# Autodesk Inventor assembly: ForeArm
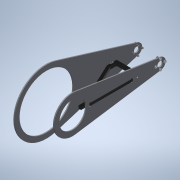
[picture p0: Inventor's stored thumbnail of the model, 180x180]
Saved by Autodesk Inventor 2020.4 (Build 244396000, 396)
## iProperties
Created: 2016-05-04
Part Number: ForeArm
Document SubType Name: Assembly
Designer: hiroaki
Mass: 49.3377 g
Surface Area: 202.128 cm^2
Volume: 30.5225 cm^3
Density: 1.61644 g/cm^3
Author: hiroaki
## Documents named in this file (5)
- C:\Users\Masato\Documents\Inventor\CIT Brains_Inventor\OpenPlatform_ver3_0 - ve4_1 branch\UpperBody\Arm\ForeArm.iam
- C:\Users\Masato\Documents\Inventor\CIT Brains_Inventor\OpenPlatform_ver3_0 - ve4_1 branch\UpperBody\Arm\ForeArm_outside_frame.ipt
- C:\Users\Masato\Documents\Inventor\CIT Brains_Inventor\OpenPlatform_ver3_0 - ve4_1 branch\UpperBody\Arm\ForeArm_diagonal.ipt
- C:\Users\Masato\Documents\Inventor\CIT Brains_Inventor\OpenPlatform_ver3_0 - ve4_1 branch\UpperBody\Arm\ForeArm_inside_frame.ipt
- C:\Users\Masato\Documents\Inventor\CIT Brains_Inventor\OpenPlatform_ver3_0 - ve4_1 branch\Ready_Made\Screw\M2_6-6.ipt
## Components (11 placed, 4 different names)
1. ForeArm_diagonal:1 — メイト:1, メイト:2, フラッシュ:1, 挿入:3, 挿入:4, 挿入:5, 挿入:6
2. ForeArm_outside_frame:1 — 挿入:3, 挿入:4, 挿入:13, 挿入:14, 挿入:15, 挿入:16
3. ForeArm_inside_frame:1 — 挿入:5, 挿入:6, 挿入:17, 挿入:18, 挿入:19, 挿入:20
4. M2_6-6:1 — 挿入:16
5. M2_6-6:2 — 挿入:17
6. M2_6-6:3 — 挿入:18
7. M2_6-6:4 — 挿入:19
8. M2_6-6:5 — 挿入:20
9. M2_6-6:6 — 挿入:13
10. M2_6-6:7 — 挿入:14
11. M2_6-6:8 — 挿入:15
## Relationships (15: Insert 12, Mate 2, Flush 1)
- メイト:1 [Mate]: ForeArm_diagonal:1
- メイト:2 [Mate]: ForeArm_diagonal:1
- フラッシュ:1 [Flush]: ForeArm_diagonal:1
- 挿入:3 [Insert]: ForeArm_diagonal:1 ↔ ForeArm_outside_frame:1
- 挿入:4 [Insert]: ForeArm_diagonal:1 ↔ ForeArm_outside_frame:1
- 挿入:5 [Insert]: ForeArm_diagonal:1 ↔ ForeArm_inside_frame:1
- 挿入:6 [Insert]: ForeArm_diagonal:1 ↔ ForeArm_inside_frame:1
- 挿入:13 [Insert]: ForeArm_outside_frame:1 ↔ M2_6-6:6
- 挿入:14 [Insert]: ForeArm_outside_frame:1 ↔ M2_6-6:7
- 挿入:15 [Insert]: ForeArm_outside_frame:1 ↔ M2_6-6:8
- 挿入:16 [Insert]: ForeArm_outside_frame:1 ↔ M2_6-6:1
- 挿入:17 [Insert]: ForeArm_inside_frame:1 ↔ M2_6-6:2
- 挿入:18 [Insert]: ForeArm_inside_frame:1 ↔ M2_6-6:3
- 挿入:19 [Insert]: ForeArm_inside_frame:1 ↔ M2_6-6:4
- 挿入:20 [Insert]: ForeArm_inside_frame:1 ↔ M2_6-6:5
